# Autodesk Inventor assembly: ArcadeController
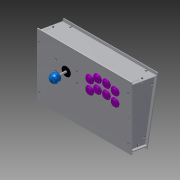
[picture p0: Inventor's stored thumbnail of the model, 180x180]
Saved by Autodesk Inventor 2013 (Build 170138000, 138)
## iProperties
Created: 2013-02-02
Part Number: ArcadeController
Document SubType Name: Assembly
Designer: xylzlyx
Author: xylzlyx
## Documents named in this file (12)
- C:\dev\pewpew\assemblies\ArcadeController.iam
- C:\dev\pewpew\parts\Panel_top.ipt
- C:\dev\pewpew\parts\Panel_bottom.ipt
- C:\dev\pewpew\parts\JLF-TP-8YT_body.ipt
- C:\dev\pewpew\parts\JLF-TP-8YT_ball.ipt
- C:\dev\pewpew\parts\JLF-TP-8YT_ring.ipt
- C:\dev\pewpew\parts\OBSF-30-B_button.ipt
- C:\dev\pewpew\assemblies\ArcadeController\Design Accelerator\Bolted Connection1.iam
- C:\dev\pewpew\parts\Panel_back.ipt
- C:\dev\pewpew\parts\Panel_front.ipt
- C:\dev\pewpew\parts\Panel_side.ipt
- C:\Users\xylzlyx\Documents\Inventor\Content Center Files\R2013\en-US\ANSI B18.3(05)\ANSI B18.3 - 6-32 UNC - 0.5(31).ipt
## Components (34 placed, 11 different names)
1. TopPanel:1 — Flush:1, Flush:2, Insert:1, Insert:2, Insert:4, Insert:5, Insert:6, Insert:7, Insert:8, Insert:9, Insert:10, Insert:11, Insert:12, Mate:1, Mate:2, Mate:6, Mate:10, Insert:15, Insert:26, Insert:27, Insert:29
2. BottomPanel:1 — Flush:1, Flush:2, Mate:3, Flush:3, Flush:4, Flush:5, Flush:6, Flush:8, Flush:9, Mate:4, Mate:5, Flush:10, Flush:12, Flush:13, Mate:8, Flush:14, Mate:13, Insert:17, Insert:18, Insert:19, Insert:20, Insert:21, Insert:22, Insert:23, Insert:24
3. JLF-TP-8YT_body:1 — Insert:1, Insert:2, Insert:3, Mate:3
4. JoystickBall:1 — Insert:3
5. JoystickCover:1 — Insert:4
6. OBSF-30-B_button:1 — Insert:5
7. OBSF-30-B_button:2 — Insert:6
8. OBSF-30-B_button:3 — Insert:7
9. OBSF-30-B_button:4 — Insert:8
10. OBSF-30-B_button:5 — Insert:9
11. OBSF-30-B_button:6 — Insert:10
12. OBSF-30-B_button:7 — Insert:11
13. OBSF-30-B_button:8 — Insert:12
14. Bolted Connection:1 [sub-assembly] — Mate:1, Mate:2
15. Panel_back:1 — Flush:3, Flush:4, Mate:5, Flush:10, Mate:11, Mate:12, Insert:13, Insert:28
16. Panel_front:1 — Flush:5, Flush:6, Flush:12, Mate:9, Flush:14, Mate:13, Insert:16, Insert:25
17. Panel_side:1 — Flush:8, Flush:9, Mate:4, Mate:6, Mate:12
18. Panel_side:2 — Flush:13, Mate:8, Mate:9, Mate:10, Mate:11
19. Hexagon Socket Head Cap Screw - Inch No. 6 - 32 UNC - 1/2:1 — Insert:13
20. Hexagon Socket Head Cap Screw - Inch No. 6 - 32 UNC - 1/2:3 — Insert:15
21. Hexagon Socket Head Cap Screw - Inch No. 6 - 32 UNC - 1/2:4 — Insert:16
22. Hexagon Socket Head Cap Screw - Inch No. 6 - 32 UNC - 1/2:5 — Insert:17
23. Hexagon Socket Head Cap Screw - Inch No. 6 - 32 UNC - 1/2:6 — Insert:20
24. Hexagon Socket Head Cap Screw - Inch No. 6 - 32 UNC - 1/2:7 — Insert:18
25. Hexagon Socket Head Cap Screw - Inch No. 6 - 32 UNC - 1/2:8 — Insert:19
26. Hexagon Socket Head Cap Screw - Inch No. 6 - 32 UNC - 1/2:9 — Insert:21
27. Hexagon Socket Head Cap Screw - Inch No. 6 - 32 UNC - 1/2:10 — Insert:23
28. Hexagon Socket Head Cap Screw - Inch No. 6 - 32 UNC - 1/2:11 — Insert:22
29. Hexagon Socket Head Cap Screw - Inch No. 6 - 32 UNC - 1/2:12 — Insert:25
30. Hexagon Socket Head Cap Screw - Inch No. 6 - 32 UNC - 1/2:13 — Insert:26
31. Hexagon Socket Head Cap Screw - Inch No. 6 - 32 UNC - 1/2:14 — Insert:24
32. Hexagon Socket Head Cap Screw - Inch No. 6 - 32 UNC - 1/2:15 — Insert:27
33. Hexagon Socket Head Cap Screw - Inch No. 6 - 32 UNC - 1/2:16 — Insert:28
34. Hexagon Socket Head Cap Screw - Inch No. 6 - 32 UNC - 1/2:17 — Insert:29
## Relationships (52: Insert 28, Flush 12, Mate 12)
- Flush:1: TopPanel:1 ↔ BottomPanel:1
- Flush:2: TopPanel:1 ↔ BottomPanel:1
- Insert:1: TopPanel:1 ↔ JLF-TP-8YT_body:1
- Insert:2: TopPanel:1 ↔ JLF-TP-8YT_body:1
- Insert:3: JLF-TP-8YT_body:1 ↔ JoystickBall:1
- Insert:4: TopPanel:1 ↔ JoystickCover:1
- Insert:5: TopPanel:1 ↔ OBSF-30-B_button:1
- Insert:6: TopPanel:1 ↔ OBSF-30-B_button:2
- Insert:7: TopPanel:1 ↔ OBSF-30-B_button:3
- Insert:8: TopPanel:1 ↔ OBSF-30-B_button:4
- Insert:9: TopPanel:1 ↔ OBSF-30-B_button:5
- Insert:10: TopPanel:1 ↔ OBSF-30-B_button:6
- Insert:11: TopPanel:1 ↔ OBSF-30-B_button:7
- Insert:12: TopPanel:1 ↔ OBSF-30-B_button:8
- Mate:1: TopPanel:1 ↔ Bolted Connection:1
- Mate:2: TopPanel:1 ↔ Bolted Connection:1
- Mate:3 (44.45 mm): BottomPanel:1 ↔ JLF-TP-8YT_body:1
- Flush:3: BottomPanel:1 ↔ Panel_back:1
- Flush:4 (-12.7 mm): BottomPanel:1 ↔ Panel_back:1
- Flush:5: BottomPanel:1 ↔ Panel_front:1
- Flush:6 (-9.525 mm): BottomPanel:1 ↔ Panel_front:1
- Flush:8 (-9.525 mm): BottomPanel:1 ↔ Panel_side:1
- Flush:9 (9.525 mm): BottomPanel:1 ↔ Panel_side:1
- Mate:4: BottomPanel:1 ↔ Panel_side:1
- Mate:5: BottomPanel:1 ↔ Panel_back:1
- Flush:10: BottomPanel:1 ↔ Panel_back:1
- Mate:6: TopPanel:1 ↔ Panel_side:1
- Flush:12 (9.525 mm): BottomPanel:1 ↔ Panel_front:1
- Flush:13 (9.525 mm): BottomPanel:1 ↔ Panel_side:2
- Mate:8: BottomPanel:1 ↔ Panel_side:2
- Mate:9: Panel_front:1 ↔ Panel_side:2
- Mate:10: TopPanel:1 ↔ Panel_side:2
- Mate:11: Panel_back:1 ↔ Panel_side:2
- Mate:12: Panel_back:1 ↔ Panel_side:1
- Flush:14: BottomPanel:1 ↔ Panel_front:1
- Mate:13: BottomPanel:1 ↔ Panel_front:1
- Insert:13: Panel_back:1 ↔ Hexagon Socket Head Cap Screw - Inch No. 6 - 32 UNC - 1/2:1
- Insert:15: TopPanel:1 ↔ Hexagon Socket Head Cap Screw - Inch No. 6 - 32 UNC - 1/2:3
- Insert:16: Panel_front:1 ↔ Hexagon Socket Head Cap Screw - Inch No. 6 - 32 UNC - 1/2:4
- Insert:17: BottomPanel:1 ↔ Hexagon Socket Head Cap Screw - Inch No. 6 - 32 UNC - 1/2:5
- Insert:18: BottomPanel:1 ↔ Hexagon Socket Head Cap Screw - Inch No. 6 - 32 UNC - 1/2:7
- Insert:19: BottomPanel:1 ↔ Hexagon Socket Head Cap Screw - Inch No. 6 - 32 UNC - 1/2:8
- Insert:20: BottomPanel:1 ↔ Hexagon Socket Head Cap Screw - Inch No. 6 - 32 UNC - 1/2:6
- Insert:21: BottomPanel:1 ↔ Hexagon Socket Head Cap Screw - Inch No. 6 - 32 UNC - 1/2:9
- Insert:22: BottomPanel:1 ↔ Hexagon Socket Head Cap Screw - Inch No. 6 - 32 UNC - 1/2:11
- Insert:23: BottomPanel:1 ↔ Hexagon Socket Head Cap Screw - Inch No. 6 - 32 UNC - 1/2:10
- Insert:24: BottomPanel:1 ↔ Hexagon Socket Head Cap Screw - Inch No. 6 - 32 UNC - 1/2:14
- Insert:25: Panel_front:1 ↔ Hexagon Socket Head Cap Screw - Inch No. 6 - 32 UNC - 1/2:12
- Insert:26: TopPanel:1 ↔ Hexagon Socket Head Cap Screw - Inch No. 6 - 32 UNC - 1/2:13
- Insert:27: TopPanel:1 ↔ Hexagon Socket Head Cap Screw - Inch No. 6 - 32 UNC - 1/2:15
- Insert:28: Panel_back:1 ↔ Hexagon Socket Head Cap Screw - Inch No. 6 - 32 UNC - 1/2:16
- Insert:29: TopPanel:1 ↔ Hexagon Socket Head Cap Screw - Inch No. 6 - 32 UNC - 1/2:17
